# Autodesk Inventor assembly: Koruza 1
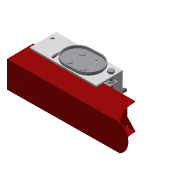
[picture p0: Inventor's stored thumbnail of the model, 180x180]
Saved by Autodesk Inventor 2015 (Build 190159000, 159)
## iProperties
Created: 2015-01-18
Part Number: Koruza 1
Document SubType Name: Assembly
Designer: Michal
Author: Michal
## Documents named in this file (17)
- C:\Users\Michal\Desktop\Michal\Prace\koruza\Koruza 1.iam
- C:\Users\Michal\Desktop\Michal\Prace\koruza\Case.ipt
- C:\Users\Michal\Desktop\Michal\Prace\koruza\U-profil 100x40 - pod case.ipt
- C:\Users\Michal\Desktop\Michal\Prace\koruza\L profil 100x100 základní.ipt
- C:\Users\Michal\Desktop\Michal\Prace\koruza\ISO 4035 - M12ISO.ipt
- C:\Users\Michal\Desktop\Michal\Prace\koruza\Šroub M12x160.ipt
- C:\Users\Michal\Desktop\Michal\Prace\koruza\DIN 127 - A 12.ipt
- C:\Users\Michal\Desktop\Michal\Prace\koruza\ANSI B18.16.3M - Property Class 5 and 10 - Metric M12 x 1.75 Typ kovu.ipt
- C:\Users\Michal\Desktop\Michal\Prace\koruza\DIN 444 - A - M12 x 55 12.ipt
- C:\Users\Michal\Desktop\Michal\Prace\koruza\Šroub M4x10.ipt
- C:\Users\Michal\Desktop\Michal\Prace\koruza\ISO 4032 - M4ISO.ipt
- C:\Users\Michal\Desktop\Michal\Prace\koruza\Anténní držák.ipt
- C:\Users\Michal\Desktop\Michal\Prace\koruza\ISO 4032 - M8ISO.ipt
- C:\Users\Michal\Desktop\Michal\Prace\koruza\ISO 7089 - 10 - 140 HV(1).ipt
- C:\Users\Michal\Desktop\Michal\Prace\koruza\Šroub M8x24.ipt
- C:\Users\Michal\Desktop\Michal\Prace\koruza\Šroub M10x70.ipt
- C:\Users\Michal\Desktop\Michal\Prace\koruza\ISO 4035 - M10ISO.ipt
## Components (32 placed, 16 different names)
1. Case:1 — Proti sobě:1, Proti sobě:2, Proti sobě:3, Proti sobě:4, Proti sobě:30, Proti sobě:31, Proti sobě:35, Proti sobě:67, Proti sobě:68
2. U-profil 100x40 - pod case:1 — Proti sobě:1, Proti sobě:2, Proti sobě:3, Proti sobě:5, Proti sobě:6, Proti sobě:11, Proti sobě:13, Proti sobě:33, Proti sobě:34, Proti sobě:37, Proti sobě:65, Proti sobě:69, Proti sobě:71
3. L profil 100x100 základní:1 — Proti sobě:4, Proti sobě:5, Proti sobě:7, Proti sobě:9, Proti sobě:21, Proti sobě:25, Proti sobě:29, Proti sobě:39, Proti sobě:40, Proti sobě:54, Proti sobě:56, Proti sobě:58, Proti sobě:66
4. Šroub M12x160:1 — Proti sobě:6, Proti sobě:7, Proti sobě:8, Proti sobě:10, Proti sobě:12, Proti sobě:20, Proti sobě:22, Proti sobě:26, Proti sobě:65, Proti sobě:66
5. ISO 4035 - M12ISO:1 — Proti sobě:12, Proti sobě:13
6. ISO 4035 - M12ISO:3 — Proti sobě:10, Proti sobě:11
7. ANSI B18.16.3M - Property Class 5 and 10 - Metric M12 x 1.75 Typ kovu:1 — Proti sobě:8, Proti sobě:9
8. DIN 444 - A - M12 x 55 12:1 — Proti sobě:20, Proti sobě:21, Proti sobě:23, Proti sobě:24, Proti sobě:27, Proti sobě:28
9. ISO 4035 - M12ISO:4 — Proti sobě:24, Proti sobě:25
10. ISO 4035 - M12ISO:5 — Proti sobě:22, Proti sobě:23
11. ISO 4035 - M12ISO:6 — Proti sobě:26, Proti sobě:27
12. ISO 4035 - M12ISO:7 — Proti sobě:28, Proti sobě:29
13. Šroub M4x10:1 — Proti sobě:34, Proti sobě:35, Proti sobě:36
14. Šroub M4x10:2 — Proti sobě:30, Proti sobě:31, Proti sobě:32
15. ISO 4032 - M4ISO:1 — Proti sobě:32, Proti sobě:33
16. ISO 4032 - M4ISO:2 — Proti sobě:36, Proti sobě:37
17. Anténní držák:1 — Proti sobě:39, Proti sobě:40, Proti sobě:41, Proti sobě:42, Proti sobě:45, Proti sobě:46, Proti sobě:49, Proti sobě:50
18. ISO 4032 - M8ISO:1 — Proti sobě:63, Proti sobě:64
19. ISO 4032 - M8ISO:2 — Proti sobě:61, Proti sobě:62
20. ISO 4032 - M8ISO:3 — Proti sobě:59, Proti sobě:60
21. ISO 7089 - 10 - 140 HV(1):1 — Proti sobě:41, Proti sobě:42, Proti sobě:43, Proti sobě:44
22. ISO 7089 - 10 - 140 HV(1):2 — Proti sobě:49, Proti sobě:50, Proti sobě:51, Proti sobě:52
23. ISO 7089 - 10 - 140 HV(1):3 — Proti sobě:45, Proti sobě:46, Proti sobě:47, Proti sobě:48
24. ISO 7089 - 10 - 140 HV(1):4 — Proti sobě:55, Proti sobě:56, Proti sobě:64
25. ISO 7089 - 10 - 140 HV(1):5 — Proti sobě:53, Proti sobě:54, Proti sobě:62
26. ISO 7089 - 10 - 140 HV(1):6 — Proti sobě:57, Proti sobě:58, Proti sobě:60
27. Šroub M8x24:1 — Proti sobě:51, Proti sobě:52, Proti sobě:57, Proti sobě:59
28. Šroub M8x24:2 — Proti sobě:47, Proti sobě:48, Proti sobě:53, Proti sobě:61
29. Šroub M8x24:3 — Proti sobě:43, Proti sobě:44, Proti sobě:55, Proti sobě:63
30. Šroub M10x70:1 — Proti sobě:67, Proti sobě:68, Proti sobě:69, Proti sobě:70, Proti sobě:72
31. DIN 127 - A 12:1 — Proti sobě:70, Proti sobě:71, Proti sobě:73
32. ISO 4035 - M10ISO:3 — Proti sobě:72, Proti sobě:73
## Relationships (66: Mate 66)
- Proti sobě:1 [Mate]: Case:1 ↔ U-profil 100x40 - pod case:1
- Proti sobě:2 [Mate]: Case:1 ↔ U-profil 100x40 - pod case:1
- Proti sobě:3 [Mate]: Case:1 ↔ U-profil 100x40 - pod case:1
- Proti sobě:4 [Mate] (25 mm): Case:1 ↔ L profil 100x100 základní:1
- Proti sobě:5 [Mate]: U-profil 100x40 - pod case:1 ↔ L profil 100x100 základní:1
- Proti sobě:6 [Mate]: U-profil 100x40 - pod case:1 ↔ Šroub M12x160:1
- Proti sobě:7 [Mate]: L profil 100x100 základní:1 ↔ Šroub M12x160:1
- Proti sobě:8 [Mate]: Šroub M12x160:1 ↔ ANSI B18.16.3M - Property Class 5 and 10 - Metric M12 x 1.75 Typ kovu:1
- Proti sobě:9 [Mate]: L profil 100x100 základní:1 ↔ ANSI B18.16.3M - Property Class 5 and 10 - Metric M12 x 1.75 Typ kovu:1
- Proti sobě:10 [Mate]: Šroub M12x160:1 ↔ ISO 4035 - M12ISO:3
- Proti sobě:11 [Mate]: U-profil 100x40 - pod case:1 ↔ ISO 4035 - M12ISO:3
- Proti sobě:12 [Mate]: Šroub M12x160:1 ↔ ISO 4035 - M12ISO:1
- Proti sobě:13 [Mate]: U-profil 100x40 - pod case:1 ↔ ISO 4035 - M12ISO:1
- Proti sobě:20 [Mate]: Šroub M12x160:1 ↔ DIN 444 - A - M12 x 55 12:1
- Proti sobě:21 [Mate]: L profil 100x100 základní:1 ↔ DIN 444 - A - M12 x 55 12:1
- Proti sobě:22 [Mate]: Šroub M12x160:1 ↔ ISO 4035 - M12ISO:5
- Proti sobě:23 [Mate]: DIN 444 - A - M12 x 55 12:1 ↔ ISO 4035 - M12ISO:5
- Proti sobě:24 [Mate]: DIN 444 - A - M12 x 55 12:1 ↔ ISO 4035 - M12ISO:4
- Proti sobě:25 [Mate]: L profil 100x100 základní:1 ↔ ISO 4035 - M12ISO:4
- Proti sobě:26 [Mate]: Šroub M12x160:1 ↔ ISO 4035 - M12ISO:6
- Proti sobě:27 [Mate]: DIN 444 - A - M12 x 55 12:1 ↔ ISO 4035 - M12ISO:6
- Proti sobě:28 [Mate]: DIN 444 - A - M12 x 55 12:1 ↔ ISO 4035 - M12ISO:7
- Proti sobě:29 [Mate]: L profil 100x100 základní:1 ↔ ISO 4035 - M12ISO:7
- Proti sobě:30 [Mate]: Case:1 ↔ Šroub M4x10:2
- Proti sobě:31 [Mate]: Case:1 ↔ Šroub M4x10:2
- Proti sobě:32 [Mate]: Šroub M4x10:2 ↔ ISO 4032 - M4ISO:1
- Proti sobě:33 [Mate]: U-profil 100x40 - pod case:1 ↔ ISO 4032 - M4ISO:1
- Proti sobě:34 [Mate]: U-profil 100x40 - pod case:1 ↔ Šroub M4x10:1
- Proti sobě:35 [Mate]: Case:1 ↔ Šroub M4x10:1
- Proti sobě:36 [Mate]: Šroub M4x10:1 ↔ ISO 4032 - M4ISO:2
- Proti sobě:37 [Mate]: U-profil 100x40 - pod case:1 ↔ ISO 4032 - M4ISO:2
- Proti sobě:39 [Mate]: L profil 100x100 základní:1 ↔ Anténní držák:1
- Proti sobě:40 [Mate]: L profil 100x100 základní:1 ↔ Anténní držák:1
- Proti sobě:41 [Mate]: Anténní držák:1 ↔ ISO 7089 - 10 - 140 HV(1):1
- Proti sobě:42 [Mate]: Anténní držák:1 ↔ ISO 7089 - 10 - 140 HV(1):1
- Proti sobě:43 [Mate]: ISO 7089 - 10 - 140 HV(1):1 ↔ Šroub M8x24:3
- Proti sobě:44 [Mate]: ISO 7089 - 10 - 140 HV(1):1 ↔ Šroub M8x24:3
- Proti sobě:45 [Mate]: Anténní držák:1 ↔ ISO 7089 - 10 - 140 HV(1):3
- Proti sobě:46 [Mate]: Anténní držák:1 ↔ ISO 7089 - 10 - 140 HV(1):3
- Proti sobě:47 [Mate]: ISO 7089 - 10 - 140 HV(1):3 ↔ Šroub M8x24:2
- Proti sobě:48 [Mate]: ISO 7089 - 10 - 140 HV(1):3 ↔ Šroub M8x24:2
- Proti sobě:49 [Mate]: Anténní držák:1 ↔ ISO 7089 - 10 - 140 HV(1):2
- Proti sobě:50 [Mate]: Anténní držák:1 ↔ ISO 7089 - 10 - 140 HV(1):2
- Proti sobě:51 [Mate]: ISO 7089 - 10 - 140 HV(1):2 ↔ Šroub M8x24:1
- Proti sobě:52 [Mate]: ISO 7089 - 10 - 140 HV(1):2 ↔ Šroub M8x24:1
- Proti sobě:53 [Mate]: ISO 7089 - 10 - 140 HV(1):5 ↔ Šroub M8x24:2
- Proti sobě:54 [Mate]: L profil 100x100 základní:1 ↔ ISO 7089 - 10 - 140 HV(1):5
- Proti sobě:55 [Mate]: ISO 7089 - 10 - 140 HV(1):4 ↔ Šroub M8x24:3
- Proti sobě:56 [Mate]: L profil 100x100 základní:1 ↔ ISO 7089 - 10 - 140 HV(1):4
- Proti sobě:57 [Mate]: ISO 7089 - 10 - 140 HV(1):6 ↔ Šroub M8x24:1
- Proti sobě:58 [Mate]: L profil 100x100 základní:1 ↔ ISO 7089 - 10 - 140 HV(1):6
- Proti sobě:59 [Mate]: ISO 4032 - M8ISO:3 ↔ Šroub M8x24:1
- Proti sobě:60 [Mate]: ISO 4032 - M8ISO:3 ↔ ISO 7089 - 10 - 140 HV(1):6
- Proti sobě:61 [Mate]: ISO 4032 - M8ISO:2 ↔ Šroub M8x24:2
- Proti sobě:62 [Mate]: ISO 4032 - M8ISO:2 ↔ ISO 7089 - 10 - 140 HV(1):5
- Proti sobě:63 [Mate]: ISO 4032 - M8ISO:1 ↔ Šroub M8x24:3
- Proti sobě:64 [Mate]: ISO 4032 - M8ISO:1 ↔ ISO 7089 - 10 - 140 HV(1):4
- Proti sobě:65 [Mate]: U-profil 100x40 - pod case:1 ↔ Šroub M12x160:1
- Proti sobě:66 [Mate]: L profil 100x100 základní:1 ↔ Šroub M12x160:1
- Proti sobě:67 [Mate]: Case:1 ↔ Šroub M10x70:1
- Proti sobě:68 [Mate]: Case:1 ↔ Šroub M10x70:1
- Proti sobě:69 [Mate]: U-profil 100x40 - pod case:1 ↔ Šroub M10x70:1
- Proti sobě:70 [Mate]: Šroub M10x70:1 ↔ DIN 127 - A 12:1
- Proti sobě:71 [Mate]: U-profil 100x40 - pod case:1 ↔ DIN 127 - A 12:1
- Proti sobě:72 [Mate]: Šroub M10x70:1 ↔ ISO 4035 - M10ISO:3
- Proti sobě:73 [Mate]: DIN 127 - A 12:1 ↔ ISO 4035 - M10ISO:3
